# Autodesk Inventor assembly: C-SCSBNAW12-16
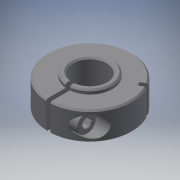
[picture p0: Inventor's stored thumbnail of the model, 180x180]
Saved by Autodesk Inventor 2019 (Build 230136000, 136)
## iProperties
Category: PARTsolutions
Company: MISUMI
Created: 2023-11-30
Part Number: C-SCSBNAW12-16
Catalog Web Link: www.cadenas.de
Description: C-SCSBNAW-Economy Shaft Collars - Slit
Vendor: MISUMI
Document SubType Name: Assembly
Designer: psAdmin
Manufacturer: MISUMI
Mass: 5.72648 g
Surface Area: 32.6924 cm^2
Volume: 5.72648 cm^3
Density: 1 g/cm^3
Title: C-SCSBNAW12-16
Author: Cadenas PARTsolutions
Comments: Economy Shaft Collars - Slit
PSOL_IDENT_0: {$CADENAS_DATA/23d-libs/misumi/metric/03_set_collars/c_scsbnaw_asmtab.prj},185 {VTYP=3D},{STYP=ASSTA
PSOL_IDENT_1: B},{NB=C-SCSBNAW12-16},{LINA=C-SCSBNAW12-16},{NN=C-SCSBNAW},{DATE=12.09.2022 02:02:40},{GEOMDATE=01.
PSOL_IDENT_2: 07.2022 02:59:35},{VERSION=},{LINEID=70},{WBVAR=},{WBNUMERIC=}  {NB=C-SCSBNAW12-16},{LINA=C-SCSBNAW1
PSOL_IDENT_3: 2-16},{KT=DUMMY},{PN=C-SCSBNAW12-16},{TYPE=C-SCSBNAW},{D=12},{DSS=16},{BB=10},{B=11.5},{D1=30},{M=M4
PSOL_IDENT_4: },{THMD=4},{DD=4.5},{H=7.5},{X=10.0},{Y=5},{W=1.5},{C=0.5},{WL=2.3},{L=12},{PPATH=c_scsbnaw/c_scsbna
PSOL_IDENT_5: w_asmtpl.prj}
NB: C-SCSBNAW12-16
NN: C-SCSBNAW
NT: Economy Shaft Collars - Slit Bearing Inner Mount
NBSYN: $PN.
LINA: C-SCSBNAW12-16
CATALOG: Misumi
PN: C-SCSBNAW12-16
D: 12
DSS: 16
BB: 10
B: 11.5
D1: 30
M: M4
DD: 4.5
H: 7.5
X: 10
Y: 5
W: 1.5
C: 0.5
SUPPLIER: MISUMI
ARTICLENO: C-SCSBNAW12-16
BOMINFO: C-SCSBNAW12-16
CREATOR: CADENAS GmbH
## Documents named in this file (3)
- e:\temp\worker_COMMON_2\temp\tmp_5112_262_UA7hW\format_0\C-SCSBNAW12-16.iam
- e:\temp\worker_COMMON_2\temp\tmp_5112_262_UA7hW\format_0\C-SCSBNAW12-16_b.ipt
- e:\temp\worker_COMMON_2\temp\tmp_5112_262_UA7hW\format_0\Slotted head cap screw ISO 4762 - M4x12.ipt
## Components (2 placed, 2 different names)
1. C-SCSBNAW12-16_b:1 — body_screw_Z@1 <-> IP1_Z@2
2. Slotted head cap screw ISO 4762 - M4x12:1 — body_screw_Z@1 <-> IP1_Z@2
## Relationships (1: Mate 1)
- body_screw_Z@1 <-> IP1_Z@2 [Mate]: C-SCSBNAW12-16_b:1 ↔ Slotted head cap screw ISO 4762 - M4x12:1
